# Autodesk Inventor assembly: BREEZE-S04
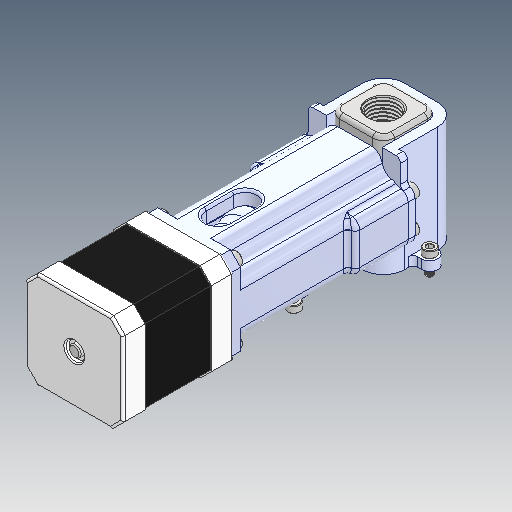
[picture p0: Inventor's stored thumbnail of the model, 512x512]
Saved by Autodesk Inventor 2020 (Build 240168000, 168)
## iProperties
Created: 2020-04-12
Part Number: BREEZE-S04
Document SubType Name: Assembly
Designer: John K
Description: STEPER ASSEMBLY
Author: John K
## Documents named in this file (9)
- C:\GrabCAD\MTL Ventilator Design\BREEZE\Subassemblies\BREEZE-S04.iam
- C:\GrabCAD\MTL Ventilator Design\BREEZE\Commercial Parts\McMaster\Needle Valve.ipt
- C:\GrabCAD\MTL Ventilator Design\BREEZE\Manufactured Parts\BREEZE-M15.ipt
- C:\GrabCAD\MTL Ventilator Design\BREEZE\Manufactured Parts\BREEZE-M17.ipt
- C:\GrabCAD\MTL Ventilator Design\BREEZE\Manufactured Parts\BREEZE-M16.ipt
- C:\GrabCAD\MTL Ventilator Design\BREEZE\Commercial Parts\McMaster\M3 Insert.ipt
- C:\GrabCAD\MTL Ventilator Design\BREEZE\Commercial Parts\Electronics\Stepper Motor.ipt
- C:\GrabCAD\MTL Ventilator Design\BREEZE\Commercial Parts\McMaster\M3x8mm Socket.ipt
- C:\GrabCAD\MTL Ventilator Design\BREEZE\Commercial Parts\McMaster\M3x8mm Set Screw.ipt
## Components (23 placed, 8 different names)
1. Needle Valve:1 — Mate:2, Mate:3, Mate:4, Mate:5, Mate:6, Mate:7
2. BREEZE-M15:1 — Mate:7, Insert:1, Insert:2, Insert:3, Insert:4, Mate:8, Mate:9, Insert:5, Mate:10, Insert:14, Insert:16, Insert:17, Insert:18, Insert:19
3. BREEZE-M17:1 — Mate:2, Mate:3, Mate:8, Mate:9, Insert:7, Insert:8, Insert:9, Insert:10, Insert:11, Insert:12, Insert:13
4. BREEZE-M16:1 — Mate:4, Mate:5, Mate:6, Mate:11
5. M3 Insert:1 — Insert:1
6. M3 Insert:2 — Insert:2
7. M3 Insert:3 — Insert:3
8. M3 Insert:4 — Insert:4
9. Stepper Motor:1 — Insert:5, Mate:10, Mate:12
10. M3x8mm Socket:1 — Insert:7
11. M3x8mm Socket:2 — Insert:8
12. M3x8mm Socket:3 — Insert:9
13. M3x8mm Socket:4 — Insert:10
14. M3x8mm Socket:5 — Insert:11
15. M3x8mm Socket:6 — Insert:12
16. M3x8mm Socket:7 — Insert:13
17. M3 Insert:5 — Insert:14, Insert:15
18. M3x8mm Socket:8 — Insert:15
19. M3x8mm Socket:9 — Insert:16
20. M3x8mm Socket:10 — Insert:17
21. M3x8mm Socket:11 — Insert:18
22. M3x8mm Socket:12 — Insert:19
23. M3x8mm Set Screw:1 — Mate:11, Mate:12
## Relationships (29: Insert 18, Mate 11)
- Mate:2: Needle Valve:1 ↔ BREEZE-M17:1
- Mate:3: Needle Valve:1 ↔ BREEZE-M17:1
- Mate:4: Needle Valve:1 ↔ BREEZE-M16:1
- Mate:5: Needle Valve:1 ↔ BREEZE-M16:1
- Mate:6: Needle Valve:1 ↔ BREEZE-M16:1
- Mate:7: Needle Valve:1 ↔ BREEZE-M15:1
- Insert:1: BREEZE-M15:1 ↔ M3 Insert:1
- Insert:2: BREEZE-M15:1 ↔ M3 Insert:2
- Insert:3: BREEZE-M15:1 ↔ M3 Insert:3
- Insert:4: BREEZE-M15:1 ↔ M3 Insert:4
- Mate:8: BREEZE-M15:1 ↔ BREEZE-M17:1
- Mate:9: BREEZE-M15:1 ↔ BREEZE-M17:1
- Insert:5: BREEZE-M15:1 ↔ Stepper Motor:1
- Mate:10: BREEZE-M15:1 ↔ Stepper Motor:1
- Insert:7: BREEZE-M17:1 ↔ M3x8mm Socket:1
- Insert:8: BREEZE-M17:1 ↔ M3x8mm Socket:2
- Insert:9: BREEZE-M17:1 ↔ M3x8mm Socket:3
- Insert:10: BREEZE-M17:1 ↔ M3x8mm Socket:4
- Insert:11: BREEZE-M17:1 ↔ M3x8mm Socket:5
- Insert:12: BREEZE-M17:1 ↔ M3x8mm Socket:6
- Insert:13: BREEZE-M17:1 ↔ M3x8mm Socket:7
- Insert:14: BREEZE-M15:1 ↔ M3 Insert:5
- Insert:15 (4 mm): M3 Insert:5 ↔ M3x8mm Socket:8
- Insert:16: BREEZE-M15:1 ↔ M3x8mm Socket:9
- Insert:17: BREEZE-M15:1 ↔ M3x8mm Socket:10
- Insert:18: BREEZE-M15:1 ↔ M3x8mm Socket:11
- Insert:19: BREEZE-M15:1 ↔ M3x8mm Socket:12
- Mate:11: BREEZE-M16:1 ↔ M3x8mm Set Screw:1
- Mate:12 (2.5 mm): Stepper Motor:1 ↔ M3x8mm Set Screw:1
